# Autodesk Inventor assembly: ASM Z-Axis Limit Switch
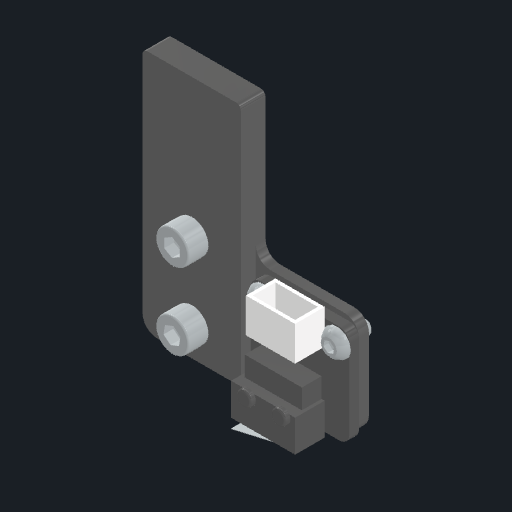
[picture p0: Inventor's stored thumbnail of the model, 512x512]
Saved by Autodesk Inventor 2024 (Build 280153000, 153)
## iProperties
Created: 2018-08-16
Part Number: ASM Z-Axis Limit Switch
Document SubType Name: Assembly
Designer: Vincent Larson
Sending System: SolidWorks 2015
Last Author: Poseidon
Last Saved: 2018-08-17
Author: Vincent Larson
## Documents named in this file (5)
- C:\Users\Vincent Larson\Downloads\Ender-3 Parts\01 MAIN ASM Ender_3\ASM Z-Axis Limit Switch.iam
- C:\Users\Vincent Larson\Downloads\Ender-3 Parts\01 MAIN ASM Ender_3\Z limit switch bracket.ipt
- C:\Users\Vincent Larson\Downloads\Ender-3 Parts\01 MAIN ASM Ender_3\limit switch.ipt
- C:\Users\Vincent Larson\Downloads\Ender-3 Parts\01 MAIN ASM Ender_3\M4X10 Socket Head Screw.ipt
- C:\Users\Vincent Larson\Downloads\Ender-3 Parts\01 MAIN ASM Ender_3\M3X6Pan Head Screw.ipt
## Components (6 placed, 4 different names)
1. Z limit switch bracket:1 — Mate:2, Mate:3, Mate:5, Mate:6, Mate:7, Mate:12
2. M4X10 Socket Head Screw:1 — Mate:5, Flush:1, Mate:7
3. M4X10 Socket Head Screw:2 — Mate:6, Flush:1
4. limit switch:1 — Mate:2, Mate:3, Mate:8, Mate:9, Mate:10, Mate:11, Mate:12
5. M3X6Pan Head Screw:3 — Mate:8, Mate:9
6. M3X6Pan Head Screw:4 — Mate:10, Mate:11
## Relationships (11: Mate 10, Flush 1)
- Mate:2: Z limit switch bracket:1 ↔ limit switch:1
- Mate:3: Z limit switch bracket:1 ↔ limit switch:1
- Mate:5: Z limit switch bracket:1 ↔ M4X10 Socket Head Screw:1
- Mate:6: Z limit switch bracket:1 ↔ M4X10 Socket Head Screw:2
- Flush:1: M4X10 Socket Head Screw:1 ↔ M4X10 Socket Head Screw:2
- Mate:7: Z limit switch bracket:1 ↔ M4X10 Socket Head Screw:1
- Mate:8: limit switch:1 ↔ M3X6Pan Head Screw:3
- Mate:9: limit switch:1 ↔ M3X6Pan Head Screw:3
- Mate:10: limit switch:1 ↔ M3X6Pan Head Screw:4
- Mate:11: limit switch:1 ↔ M3X6Pan Head Screw:4
- Mate:12: Z limit switch bracket:1 ↔ limit switch:1
